# Autodesk Inventor assembly: 01 ASY GBK wall shield 1.1.1
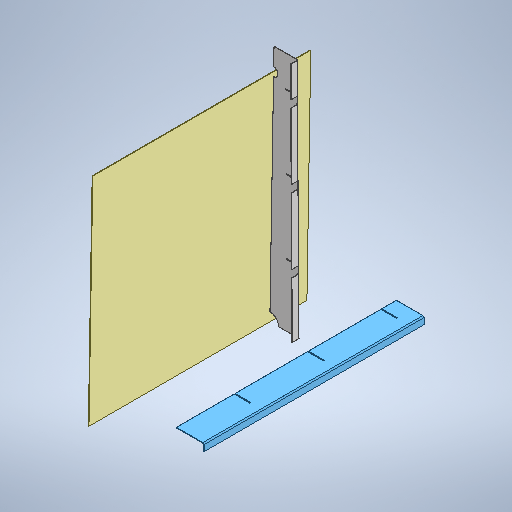
[picture p0: Inventor's stored thumbnail of the model, 512x512]
Saved by Autodesk Inventor 2026 (Build 300175000, 175)
## iProperties
Created: 2026-05-07
Part Number: 01 ASY GBK wall shield 1.1.1
Document SubType Name: Assembly
Designer: admin
Mass: 245734 g
Surface Area: 167509 cm^2
Volume: 31303.7 cm^3
Density: 7.85 g/cm^3
Author: admin
## Documents named in this file (4)
- C:\Users\pokla\Documents\Inventor\GBK-Gubkinskiy\01 ASY GBK wall shield 1.1.1.iam
- C:\Users\pokla\Documents\Inventor\GBK-Gubkinskiy\01.1 GBK shield.ipt
- C:\Users\pokla\Documents\Inventor\GBK-Gubkinskiy\01.3 GBK stringer 1.ipt
- C:\Users\pokla\Documents\Inventor\GBK-Gubkinskiy\01.2 GBK main rib.ipt
## Components (3 placed, 3 different names)
1. 01.1 GBK shield.ipt:1 — Совмещение:1, Заподлицо:1, Совмещение:2
2. 01.2 GBK main rib.ipt:1 — Совмещение:1, Заподлицо:1, Совмещение:2
3. 01.3 GBK stringer.ipt:1
## Relationships (3: Mate 2, Flush 1)
- Совмещение:1 [Mate]: 01.1 GBK shield.ipt:1 ↔ 01.2 GBK main rib.ipt:1
- Заподлицо:1 [Flush] (250 mm): 01.1 GBK shield.ipt:1 ↔ 01.2 GBK main rib.ipt:1
- Совмещение:2 [Mate]: 01.1 GBK shield.ipt:1 ↔ 01.2 GBK main rib.ipt:1
